# Autodesk Inventor assembly: Base 01
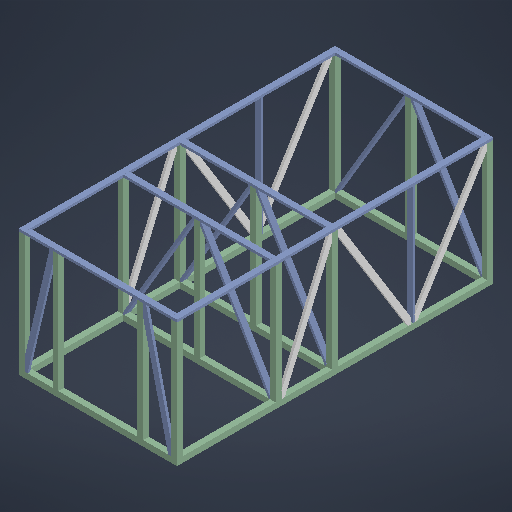
[picture p0: Inventor's stored thumbnail of the model, 512x512]
Saved by Autodesk Inventor 2026 (Build 300175000, 175)
## iProperties
Created: 2024-09-16
Part Number: Base 01
Document SubType Name: Assembly
Designer: User
Author: User
## Documents named in this file (11)
- C:\Users\trott\Documents\UofSC-ASME-Tiger-Burn-Design-2025\CAD\Body\Base 01\Base 01.iam
- C:\Users\trott\Documents\UofSC-ASME-Tiger-Burn-Design-2025\CAD\Body\Base 01\4x4x192.ipt
- C:\Users\trott\Documents\UofSC-ASME-Tiger-Burn-Design-2025\CAD\Body\Base 01\4x4x89.ipt
- C:\Users\trott\Documents\UofSC-ASME-Tiger-Burn-Design-2025\CAD\Body\Base 01\4x4x72.ipt
- C:\Users\trott\Documents\UofSC-ASME-Tiger-Burn-Design-2025\CAD\Body\Base 01\2x4x72.ipt
- C:\Users\trott\Documents\UofSC-ASME-Tiger-Burn-Design-2025\CAD\Body\Base 01\2x4x192.ipt
- C:\Users\trott\Documents\UofSC-ASME-Tiger-Burn-Design-2025\CAD\Body\Base 01\2x4x89.ipt
- C:\Users\trott\Documents\UofSC-ASME-Tiger-Burn-Design-2025\CAD\Body\Base 01\S_2x4x73.980.ipt
- C:\Users\trott\Documents\UofSC-ASME-Tiger-Burn-Design-2025\CAD\Body\Base 01\S_2x4x78.292.ipt
- C:\Users\trott\Documents\UofSC-ASME-Tiger-Burn-Design-2025\CAD\Body\Base 01\S_2x4x84.708.ipt
- C:\Users\trott\Documents\UofSC-ASME-Tiger-Burn-Design-2025\CAD\Body\Base 01\S_2x4x83.735.ipt
## Components (41 placed, 10 different names)
1. 4x4x192:1 — Mate:1, Flush:1, Flush:2, Mate:3, Flush:5, Flush:6, Flush:7, Flush:8, Flush:9, Mate:8, Mate:9, Mate:10, Mate:11, Mate:12, Mate:13, Mate:16, Flush:12, Flush:13, Flush:14, Flush:17, Flush:20, Mate:20, Flush:34, Mate:76
2. 4x4x192:2 — Mate:1, Flush:1, Flush:2, Flush:3, Mate:2, Flush:4, Mate:4, Mate:5, Mate:7, Flush:10, Flush:11, Mate:15, Mate:17, Mate:18, Flush:19, Flush:23, Flush:24, Flush:35, Mate:22, Mate:72
3. 4x4x89:1 — Flush:3, Mate:2, Flush:4, Mate:6, Flush:58, Mate:64, Mate:68
4. 4x4x89:2 — Mate:3, Flush:5, Flush:6, Flush:21, Flush:22, Flush:27
5. 4x4x89:3 — Flush:7, Mate:4, Flush:8, Flush:15, Flush:25, Flush:31
6. 4x4x89:4 — Flush:9, Mate:5, Mate:6, Mate:14, Flush:16, Flush:18, Flush:29
7. 4x4x72:1 — Mate:7, Flush:10, Flush:11, Mate:24, Flush:36, Flush:37, Mate:59, Mate:67
8. 4x4x72:12 — Mate:8, Flush:12, Flush:13, Mate:55, Mate:25, Mate:63
9. 4x4x72:13 — Mate:9, Flush:14, Flush:15, Flush:30, Mate:75
10. 4x4x72:14 — Mate:11, Mate:55, Mate:61, Mate:62
11. 4x4x72:15 — Mate:10, Flush:24, Flush:25, Mate:71
12. 4x4x72:16 — Mate:14, Flush:28, Flush:29, Mate:28, Flush:44, Mate:89, Mate:90, Mate:93, Mate:94
13. 4x4x72:17 — Mate:15, Flush:26, Flush:27, Mate:29, Flush:42, Mate:91, Mate:92, Mate:95, Mate:96
14. 4x4x72:18 — Mate:16, Flush:20, Flush:21, Mate:21, Flush:38, Flush:39, Mate:83, Mate:84
15. 4x4x72:19 — Mate:18, Flush:18, Flush:19, Flush:28, Mate:69, Mate:70, Mate:79, Mate:80
16. 4x4x72:20 — Mate:17, Flush:22, Flush:23, Flush:26, Mate:23, Mate:81, Mate:82
17. 4x4x72:21 — Mate:13, Flush:30, Flush:31, Mate:27, Flush:43, Mate:85, Mate:86, Mate:87, Mate:88
18. 4x4x72:23 — Flush:58, Mate:58, Mate:59, Mate:65, Mate:66
19. 4x4x72:22 — Mate:12, Flush:16, Flush:17, Mate:73, Mate:74, Mate:77, Mate:78
20. 2x4x72:1 — Mate:20, Flush:34, Mate:21
21. 2x4x72:2 — Flush:35, Mate:22, Mate:23
22. 2x4x192:1 — Mate:24, Flush:36, Flush:37, Mate:26, Flush:40, Flush:41, Mate:31, Symmetry:1
23. 2x4x192:2 — Mate:25, Flush:38, Flush:39, Mate:30, Mate:32, Symmetry:1
24. 2x4x89:1 — Mate:26, Flush:40, Flush:41, Mate:58
25. 2x4x89:2 — Mate:27, Mate:32, Flush:43
26. 2x4x89:3 — Mate:28, Mate:31, Flush:44
27. 2x4x89:4 — Mate:29, Flush:42, Mate:30
28. S_2x4x73.980:1 — Mate:61, Mate:62, Mate:63, Mate:64
29. S_2x4x73.980:2 — Mate:65, Mate:66, Mate:67, Mate:68
30. S_2x4x78.292:1 — Mate:69, Mate:70, Mate:71, Mate:72
31. S_2x4x78.292:2 — Mate:73, Mate:74, Mate:75, Mate:76
32. S_2x4x84.708:1 — Mate:77, Mate:78
33. S_2x4x83.735:1 — Mate:85, Mate:86
34. S_2x4x84.708:2 — Mate:79, Mate:80
35. S_2x4x84.708:3 — Mate:81, Mate:82
36. S_2x4x84.708:4 — Mate:83, Mate:84
37. S_2x4x83.735:2 — Mate:87, Mate:88
38. S_2x4x83.735:3 — Mate:89, Mate:90
39. S_2x4x83.735:4 — Mate:93, Mate:94
40. S_2x4x83.735:5 — Mate:91, Mate:92
41. S_2x4x83.735:6 — Mate:95, Mate:96
## Relationships (114: Mate 70, Flush 43, Symmetry 1)
- Mate:1 (2260.6 mm): 4x4x192:1 ↔ 4x4x192:2
- Flush:1: 4x4x192:1 ↔ 4x4x192:2
- Flush:2: 4x4x192:1 ↔ 4x4x192:2
- Flush:3: 4x4x192:2 ↔ 4x4x89:1
- Mate:2: 4x4x192:2 ↔ 4x4x89:1
- Flush:4: 4x4x192:2 ↔ 4x4x89:1
- Mate:3: 4x4x192:1 ↔ 4x4x89:2
- Flush:5: 4x4x192:1 ↔ 4x4x89:2
- Flush:6: 4x4x192:1 ↔ 4x4x89:2
- Flush:7 (1524 mm): 4x4x192:1 ↔ 4x4x89:3
- Mate:4: 4x4x192:2 ↔ 4x4x89:3
- Flush:8: 4x4x192:1 ↔ 4x4x89:3
- Flush:9: 4x4x192:1 ↔ 4x4x89:4
- Mate:5: 4x4x192:2 ↔ 4x4x89:4
- Mate:6 (2393.95 mm): 4x4x89:1 ↔ 4x4x89:4
- Mate:7: 4x4x192:2 ↔ 4x4x72:1
- Flush:10: 4x4x192:2 ↔ 4x4x72:1
- Flush:11: 4x4x192:2 ↔ 4x4x72:1
- Mate:8: 4x4x192:1 ↔ 4x4x72:12
- Mate:9: 4x4x192:1 ↔ 4x4x72:13
- Mate:10: 4x4x192:1 ↔ 4x4x72:15
- Mate:11: 4x4x192:1 ↔ 4x4x72:14
- Mate:12: 4x4x192:1 ↔ 4x4x72:22
- Mate:13: 4x4x192:1 ↔ 4x4x72:21
- Mate:14: 4x4x89:4 ↔ 4x4x72:16
- Mate:15: 4x4x192:2 ↔ 4x4x72:17
- Mate:16: 4x4x192:1 ↔ 4x4x72:18
- Mate:17: 4x4x192:2 ↔ 4x4x72:20
- Mate:18: 4x4x192:2 ↔ 4x4x72:19
- Flush:12: 4x4x192:1 ↔ 4x4x72:12
- Flush:13: 4x4x192:1 ↔ 4x4x72:12
- Flush:14: 4x4x192:1 ↔ 4x4x72:13
- Flush:15: 4x4x89:3 ↔ 4x4x72:13
- Flush:16: 4x4x89:4 ↔ 4x4x72:22
- Flush:17: 4x4x192:1 ↔ 4x4x72:22
- Flush:18: 4x4x89:4 ↔ 4x4x72:19
- Flush:19: 4x4x192:2 ↔ 4x4x72:19
- Flush:20: 4x4x192:1 ↔ 4x4x72:18
- Flush:21: 4x4x89:2 ↔ 4x4x72:18
- Flush:22: 4x4x89:2 ↔ 4x4x72:20
- Flush:23: 4x4x192:2 ↔ 4x4x72:20
- Flush:24: 4x4x192:2 ↔ 4x4x72:15
- Flush:25: 4x4x89:3 ↔ 4x4x72:15
- Flush:26 (-1174.75 mm): 4x4x72:17 ↔ 4x4x72:20
- Flush:27: 4x4x89:2 ↔ 4x4x72:17
- Flush:28 (1174.75 mm): 4x4x72:16 ↔ 4x4x72:19
- Flush:29: 4x4x89:4 ↔ 4x4x72:16
- Flush:30 (1174.75 mm): 4x4x72:13 ↔ 4x4x72:21
- Flush:31: 4x4x89:3 ↔ 4x4x72:21
- Mate:55 (-609.6 mm): 4x4x72:12 ↔ 4x4x72:14
- Mate:20: 4x4x192:1 ↔ 2x4x72:1
- Flush:34: 4x4x192:1 ↔ 2x4x72:1
- Mate:21 (-1238.25 mm): 4x4x72:18 ↔ 2x4x72:1
- Flush:35: 4x4x192:2 ↔ 2x4x72:2
- Mate:22: 4x4x192:2 ↔ 2x4x72:2
- Mate:23 (-1238.25 mm): 4x4x72:20 ↔ 2x4x72:2
- Mate:24: 4x4x72:1 ↔ 2x4x192:1
- Flush:36: 4x4x72:1 ↔ 2x4x192:1
- Flush:37: 4x4x72:1 ↔ 2x4x192:1
- Mate:25: 4x4x72:12 ↔ 2x4x192:2
- Flush:38: 4x4x72:18 ↔ 2x4x192:2
- Flush:39: 4x4x72:18 ↔ 2x4x192:2
- Mate:26: 2x4x192:1 ↔ 2x4x89:1
- Flush:40: 2x4x192:1 ↔ 2x4x89:1
- Flush:41: 2x4x192:1 ↔ 2x4x89:1
- Mate:27: 4x4x72:21 ↔ 2x4x89:2
- Mate:28: 4x4x72:16 ↔ 2x4x89:3
- Mate:29: 4x4x72:17 ↔ 2x4x89:4
- Flush:42: 4x4x72:17 ↔ 2x4x89:4
- Mate:30: 2x4x192:2 ↔ 2x4x89:4
- Mate:31: 2x4x192:1 ↔ 2x4x89:3
- Mate:32: 2x4x192:2 ↔ 2x4x89:2
- Flush:43: 4x4x72:21 ↔ 2x4x89:2
- Flush:44: 4x4x72:16 ↔ 2x4x89:3
- Symmetry:1: 2x4x192:1 ↔ 2x4x192:2
- Flush:58: 4x4x89:1 ↔ 4x4x72:23
- Mate:58: 4x4x72:23 ↔ 2x4x89:1
- Mate:59 (-609.6 mm): 4x4x72:1 ↔ 4x4x72:23
- Mate:61: 4x4x72:14 ↔ S_2x4x73.980:1
- Mate:62: 4x4x72:14 ↔ S_2x4x73.980:1
- Mate:63: 4x4x72:12 ↔ S_2x4x73.980:1
- Mate:64: 4x4x89:1 ↔ S_2x4x73.980:1
- Mate:65: 4x4x72:23 ↔ S_2x4x73.980:2
- Mate:66: 4x4x72:23 ↔ S_2x4x73.980:2
- Mate:67: 4x4x72:1 ↔ S_2x4x73.980:2
- Mate:68: 4x4x89:1 ↔ S_2x4x73.980:2
- Mate:69: 4x4x72:19 ↔ S_2x4x78.292:1
- Mate:70: 4x4x72:19 ↔ S_2x4x78.292:1
- Mate:71: 4x4x72:15 ↔ S_2x4x78.292:1
- Mate:72: 4x4x192:2 ↔ S_2x4x78.292:1
- Mate:73: 4x4x72:22 ↔ S_2x4x78.292:2
- Mate:74: 4x4x72:22 ↔ S_2x4x78.292:2
- Mate:75: 4x4x72:13 ↔ S_2x4x78.292:2
- Mate:76: 4x4x192:1 ↔ S_2x4x78.292:2
- Mate:77: 4x4x72:22 ↔ S_2x4x84.708:1
- Mate:78: 4x4x72:22 ↔ S_2x4x84.708:1
- Mate:79: 4x4x72:19 ↔ S_2x4x84.708:2
- Mate:80: 4x4x72:19 ↔ S_2x4x84.708:2
- Mate:81: 4x4x72:20 ↔ S_2x4x84.708:3
- Mate:82: 4x4x72:20 ↔ S_2x4x84.708:3
- Mate:83: 4x4x72:18 ↔ S_2x4x84.708:4
- Mate:84: 4x4x72:18 ↔ S_2x4x84.708:4
- Mate:85: 4x4x72:21 ↔ S_2x4x83.735:1
- Mate:86: 4x4x72:21 ↔ S_2x4x83.735:1
- Mate:87: 4x4x72:21 ↔ S_2x4x83.735:2
- Mate:88: 4x4x72:21 ↔ S_2x4x83.735:2
- Mate:89: 4x4x72:16 ↔ S_2x4x83.735:3
- Mate:90: 4x4x72:16 ↔ S_2x4x83.735:3
- Mate:91: 4x4x72:17 ↔ S_2x4x83.735:5
- Mate:92: 4x4x72:17 ↔ S_2x4x83.735:5
- Mate:93: 4x4x72:16 ↔ S_2x4x83.735:4
- Mate:94: 4x4x72:16 ↔ S_2x4x83.735:4
- Mate:95: 4x4x72:17 ↔ S_2x4x83.735:6
- Mate:96: 4x4x72:17 ↔ S_2x4x83.735:6
